# Autodesk Inventor assembly: Basement_And_Basement_And_First_Floor_Transition
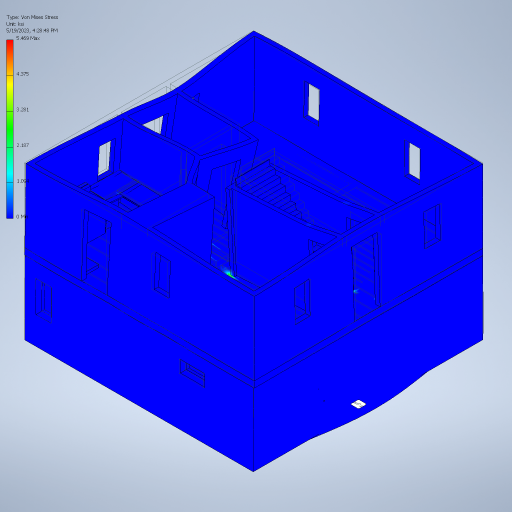
[picture p0: Inventor's stored thumbnail of the model, 512x512]
Saved by Autodesk Inventor 2024 (Build 280153000, 153)
## iProperties
Created: 2023-05-18
Part Number: Basement_And_Basement_And_First_Floor_Transition
Document SubType Name: Assembly
Designer: Tom
Author: Tom
## Documents named in this file (14)
- C:\Users\Tom\Documents\Tom_Levers_Public_Git_Repository\Inventor\Mobility\House--Finished.iam
- C:\Users\Tom\Documents\Tom_Levers_Public_Git_Repository\Inventor\Mobility\Basement\Finished_Basement.iam
- C:\Users\Tom\Documents\Tom_Levers_Public_Git_Repository\Inventor\Mobility\Finished_Basement_And_First_Floor_Transition.ipt
- C:\Users\Tom\Documents\Tom_Levers_Public_Git_Repository\Inventor\Mobility\First_Floor\First_Floor.iam
- C:\Users\Tom\Documents\Tom_Levers_Public_Git_Repository\Inventor\Mobility\First_Floor\Window_Cabinet\Window_Cabinet.iam
- C:\Users\Tom\Documents\Tom_Levers_Public_Git_Repository\Inventor\Mobility\First_Floor\Range.ipt
- C:\Users\Tom\Documents\Tom_Levers_Public_Git_Repository\Inventor\Mobility\First_Floor\Stairs_Between_First_Floor_And_Second_Floor.ipt
- C:\Users\Tom\Documents\Tom_Levers_Public_Git_Repository\Inventor\Mobility\Finished_Basement_And_Finished_Basement_And_First_Floor_Transition\AIP\FEA\ec9da2fmp.fres
- C:\Users\Tom\Documents\Tom_Levers_Public_Git_Repository\Inventor\Mobility\House--Finished\AIP\FEA\ec9da2fi8.fins
- C:\Users\Tom\Documents\Tom_Levers_Public_Git_Repository\Inventor\Mobility\House--Finished\AIP\FEA\ec9da2fj4.fsat
- C:\Users\Tom\Documents\Tom_Levers_Public_Git_Repository\Inventor\Mobility\House--Finished\AIP\FEA\ec9da2fj4.ftes
- C:\Users\Tom\Documents\Tom_Levers_Public_Git_Repository\Inventor\Mobility\House--Finished\AIP\FEA\ec9da2fj4.fwiz
- C:\Users\Tom\Documents\Tom_Levers_Public_Git_Repository\Inventor\Mobility\House--Finished\AIP\FEA\ec9da2fmo.fmsh
- C:\Users\Tom\Documents\Tom_Levers_Public_Git_Repository\Inventor\Mobility\House--Finished\AIP\FEA\ec9ngfexs.fres
## Components (6 placed, 6 different names)
1. Finished_Basement:1 [sub-assembly] — Mate:1, Flush:1, Flush:2, Flush:3, Flush:4
2. Finished_Basement_And_First_Floor_Transition:1 — Mate:1, Flush:1, Flush:2, Mate:5, Mate:7, Mate:10, Mate:11
3. First_Floor:1 [sub-assembly] — Mate:8, Mate:9, Flush:3, Mate:11, Flush:4
4. Window_Cabinet:1 [sub-assembly] — Mate:5
5. Range:1 — Mate:7
6. Stairs_Between_First_Floor_And_Second_Floor:1 — Mate:8, Mate:9, Mate:10
## Relationships (11: Mate 7, Flush 4)
- Mate:1: Finished_Basement:1 ↔ Finished_Basement_And_First_Floor_Transition:1
- Flush:1: Finished_Basement:1 ↔ Finished_Basement_And_First_Floor_Transition:1
- Flush:2 (215.9 mm): Finished_Basement:1 ↔ Finished_Basement_And_First_Floor_Transition:1
- Mate:5: Finished_Basement_And_First_Floor_Transition:1 ↔ Window_Cabinet:1
- Mate:7: Finished_Basement_And_First_Floor_Transition:1 ↔ Range:1
- Mate:8 (1244.6 mm): First_Floor:1 ↔ Stairs_Between_First_Floor_And_Second_Floor:1
- Mate:9: First_Floor:1 ↔ Stairs_Between_First_Floor_And_Second_Floor:1
- Mate:10: Finished_Basement_And_First_Floor_Transition:1 ↔ Stairs_Between_First_Floor_And_Second_Floor:1
- Flush:3: Finished_Basement:1 ↔ First_Floor:1
- Mate:11: Finished_Basement_And_First_Floor_Transition:1 ↔ First_Floor:1
- Flush:4 (215.9 mm): Finished_Basement:1 ↔ First_Floor:1
## Named parameters: sa_0 = 980.999
note: some values were not read from the file. Shown as the stored number, unit unknown: "sa_0".
